# Autodesk Inventor assembly: 4ax_plate_joint_asm
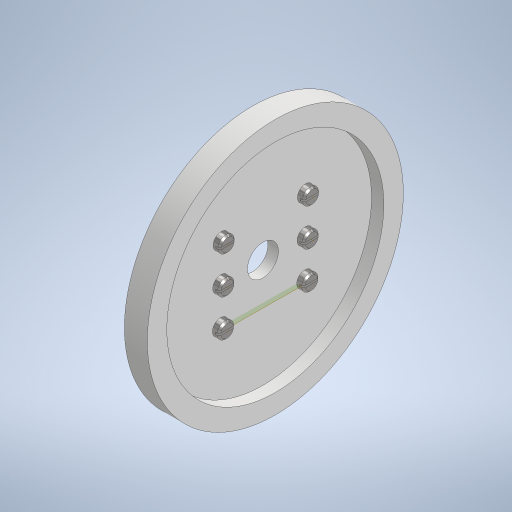
[picture p0: Inventor's stored thumbnail of the model, 512x512]
Saved by Autodesk Inventor 2024 (Build 280153000, 153)
## iProperties
Created: 2025-12-20
Part Number: 4ax_plate_joint_asm
Document SubType Name: Assembly
Designer: schar
Author: schar
## Documents named in this file (4)
- C:\Users\schar\Desktop\projectBlueprint\AMSTS\hardware\4ax_plate_joint_asm.iam
- C:\Users\schar\Desktop\projectBlueprint\AMSTS\hardware\4ax_plate_joint.ipt
- C:\Users\schar\Documents\Inventor\Content Center Files\R2024\en-US\DIN 920\DIN 920 - M5 x 10.ipt
- C:\Users\schar\Desktop\projectBlueprint\AMSTS\hardware\tnut_m5_2020.ipt
## Components (13 placed, 3 different names)
1. 4ax_plate_joint:1 — Mate:1, Mate:2, Mate:3, Mate:4, Mate:5, Mate:6, Mate:7, Mate:8, Mate:9, Mate:10, Mate:11, Mate:12, Mate:19, Mate:31, Mate:34, Mate:36, Mate:39, Mate:42
2. DIN 920 M5 x 10:1 — Mate:4, Mate:9, Mate:24, Mate:40
3. DIN 920 M5 x 10:2 — Mate:5, Mate:8, Mate:22
4. DIN 920 M5 x 10:3 — Mate:6, Mate:7, Mate:14, Mate:30
5. DIN 920 M5 x 10:4 — Mate:3, Mate:12, Mate:23, Mate:43
6. DIN 920 M5 x 10:5 — Mate:2, Mate:11, Mate:20, Mate:21, Mate:33
7. DIN 920 M5 x 10:6 — Mate:1, Mate:10, Mate:13, Mate:18
8. tnut_m5_2020:1 — Mate:17, Mate:18, Mate:19
9. tnut_m5_2020:2 — Mate:32, Mate:33, Mate:34
10. tnut_m5_2020:3 — Mate:41, Mate:42, Mate:43
11. tnut_m5_2020:4 — Mate:29, Mate:30, Mate:31
12. tnut_m5_2020:5 — Mate:35, Mate:36, Mate:37
13. tnut_m5_2020:6 — Mate:38, Mate:39, Mate:40
## Relationships (43: Mate 43)
- Mate:1: 4ax_plate_joint:1 ↔ DIN 920 M5 x 10:6
- Mate:2: 4ax_plate_joint:1 ↔ DIN 920 M5 x 10:5
- Mate:3: 4ax_plate_joint:1 ↔ DIN 920 M5 x 10:4
- Mate:4: 4ax_plate_joint:1 ↔ DIN 920 M5 x 10:1
- Mate:5: 4ax_plate_joint:1 ↔ DIN 920 M5 x 10:2
- Mate:6: 4ax_plate_joint:1 ↔ DIN 920 M5 x 10:3
- Mate:7: 4ax_plate_joint:1 ↔ DIN 920 M5 x 10:3
- Mate:8: 4ax_plate_joint:1 ↔ DIN 920 M5 x 10:2
- Mate:9: 4ax_plate_joint:1 ↔ DIN 920 M5 x 10:1
- Mate:10: 4ax_plate_joint:1 ↔ DIN 920 M5 x 10:6
- Mate:11: 4ax_plate_joint:1 ↔ DIN 920 M5 x 10:5
- Mate:12: 4ax_plate_joint:1 ↔ DIN 920 M5 x 10:4
- Mate:13: DIN 920 M5 x 10:6
- Mate:14: DIN 920 M5 x 10:3
- Mate:15
- Mate:16
- Mate:17 (-3 mm): tnut_m5_2020:1
- Mate:18: DIN 920 M5 x 10:6 ↔ tnut_m5_2020:1
- Mate:19 (0.159 mm): 4ax_plate_joint:1 ↔ tnut_m5_2020:1
- Mate:20: DIN 920 M5 x 10:5
- Mate:21: DIN 920 M5 x 10:5
- Mate:22: DIN 920 M5 x 10:2
- Mate:23: DIN 920 M5 x 10:4
- Mate:24: DIN 920 M5 x 10:1
- Mate:25
- Mate:26
- Mate:27
- Mate:28
- Mate:29 (-3 mm): tnut_m5_2020:4
- Mate:30: DIN 920 M5 x 10:3 ↔ tnut_m5_2020:4
- Mate:31 (0.159 mm): 4ax_plate_joint:1 ↔ tnut_m5_2020:4
- Mate:32 (-3 mm): tnut_m5_2020:2
- Mate:33: DIN 920 M5 x 10:5 ↔ tnut_m5_2020:2
- Mate:34 (0.159 mm): 4ax_plate_joint:1 ↔ tnut_m5_2020:2
- Mate:35 (-3 mm): tnut_m5_2020:5
- Mate:36 (0.159 mm): 4ax_plate_joint:1 ↔ tnut_m5_2020:5
- Mate:37: tnut_m5_2020:5
- Mate:38 (-3 mm): tnut_m5_2020:6
- Mate:39 (0.159 mm): 4ax_plate_joint:1 ↔ tnut_m5_2020:6
- Mate:40: DIN 920 M5 x 10:1 ↔ tnut_m5_2020:6
- Mate:41 (-3 mm): tnut_m5_2020:3
- Mate:42 (0.159 mm): 4ax_plate_joint:1 ↔ tnut_m5_2020:3
- Mate:43: DIN 920 M5 x 10:4 ↔ tnut_m5_2020:3
